# Autodesk Inventor assembly: ModulWalkaNapinajacego
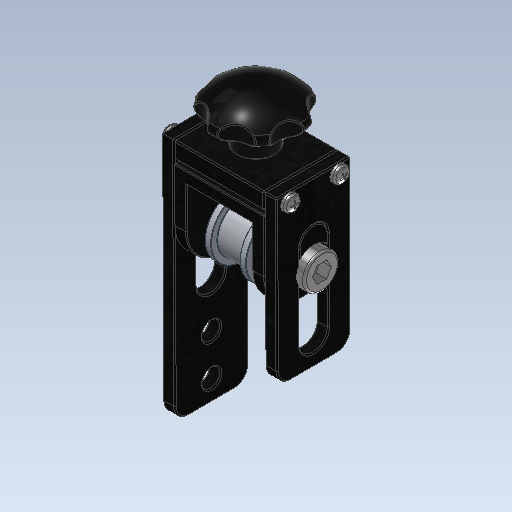
[picture p0: Inventor's stored thumbnail of the model, 512x512]
Saved by Autodesk Inventor 2020 (Build 240168000, 168)
## iProperties
Created: 2020-08-21
Part Number: ModulWalkaNapinajacego
Document SubType Name: Assembly
Designer: estee
Author: estee
## Documents named in this file (9)
- C:\Users\Hesekiel\Desktop\Equatorial-Mount-MUM\Mechanika\Moduł obrotu DEK Bartek\Prawie Gotowe\ModulWalkaNapinajacego.iam
- C:\Users\Hesekiel\Desktop\Equatorial-Mount-MUM\Mechanika\Moduł obrotu DEK Bartek\Prawie Gotowe\Ramka1.ipt
- C:\Users\Hesekiel\Desktop\Equatorial-Mount-MUM\Mechanika\Moduł obrotu DEK Bartek\Prawie Gotowe\Ramka2.ipt
- C:\Users\Hesekiel\Desktop\Equatorial-Mount-MUM\Mechanika\Moduł obrotu DEK Bartek\Prawie Gotowe\Ramka3.ipt
- C:\Users\Hesekiel\Desktop\Equatorial-Mount-MUM\Mechanika\Moduł obrotu DEK Bartek\Prawie Gotowe\Ramka4.ipt
- C:\Users\Hesekiel\Desktop\Equatorial-Mount-MUM\Mechanika\Moduł obrotu DEK Bartek\Prawie Gotowe\EN ISO 7045 - M2 x 6 - 4.8 - H(1).ipt
- C:\Users\Hesekiel\Desktop\Equatorial-Mount-MUM\Mechanika\Moduł obrotu DEK Bartek\Prawie Gotowe\ModulKolaNapinajacego.iam
- C:\Users\Hesekiel\Desktop\Equatorial-Mount-MUM\Mechanika\Moduł obrotu DEK Bartek\Prawie Gotowe\Star Knob M6 Male.ipt
- C:\Users\Hesekiel\Desktop\Equatorial-Mount-MUM\Mechanika\Moduł obrotu DEK Bartek\Prawie Gotowe\ISO 4762 - M5 x 25ISO.ipt
## Components (11 placed, 8 different names)
1. Ramka1:1 — Mate:1, Mate:2, Flush:1, Mate:3, Mate:4, Flush:2, Mate:6, Mate:19, Mate:20, Mate:21, Mate:22
2. Ramka2:1 — Mate:1, Mate:2, Flush:1, Mate:5, Mate:7, Mate:8, Mate:13, Mate:14
3. Ramka3:1 — Mate:3, Mate:4, Flush:2, Mate:9, Mate:10, Mate:11, Mate:12
4. Ramka4:1 — Mate:5, Mate:6, Mate:15, Mate:16
5. BS EN ISO 7045 H - Metric M2 x 6 - 4.8 - H:1 — Mate:7, Mate:13
6. BS EN ISO 7045 H - Metric M2 x 6 - 4.8 - H:2 — Mate:8, Mate:14
7. BS EN ISO 7045 H - Metric M2 x 6 - 4.8 - H:3 — Mate:9, Mate:11
8. BS EN ISO 7045 H - Metric M2 x 6 - 4.8 - H:4 — Mate:10, Mate:12
9. ModulKolaNapinajacego:1 [sub-assembly] — Mate:19, Mate:20
10. Star Knob M6 Male:1 — Mate:15, Mate:16
11. ISO 4762 M5 x 25:1 — Mate:21, Mate:22
## Relationships (22: Mate 20, Flush 2)
- Mate:1: Ramka1:1 ↔ Ramka2:1
- Mate:2: Ramka1:1 ↔ Ramka2:1
- Flush:1: Ramka1:1 ↔ Ramka2:1
- Mate:3: Ramka1:1 ↔ Ramka3:1
- Mate:4: Ramka1:1 ↔ Ramka3:1
- Flush:2: Ramka1:1 ↔ Ramka3:1
- Mate:5: Ramka2:1 ↔ Ramka4:1
- Mate:6: Ramka1:1 ↔ Ramka4:1
- Mate:7: Ramka2:1 ↔ BS EN ISO 7045 H - Metric M2 x 6 - 4.8 - H:1
- Mate:8: Ramka2:1 ↔ BS EN ISO 7045 H - Metric M2 x 6 - 4.8 - H:2
- Mate:9: Ramka3:1 ↔ BS EN ISO 7045 H - Metric M2 x 6 - 4.8 - H:3
- Mate:10: Ramka3:1 ↔ BS EN ISO 7045 H - Metric M2 x 6 - 4.8 - H:4
- Mate:11: Ramka3:1 ↔ BS EN ISO 7045 H - Metric M2 x 6 - 4.8 - H:3
- Mate:12: Ramka3:1 ↔ BS EN ISO 7045 H - Metric M2 x 6 - 4.8 - H:4
- Mate:13: Ramka2:1 ↔ BS EN ISO 7045 H - Metric M2 x 6 - 4.8 - H:1
- Mate:14: Ramka2:1 ↔ BS EN ISO 7045 H - Metric M2 x 6 - 4.8 - H:2
- Mate:15: Ramka4:1 ↔ Star Knob M6 Male:1
- Mate:16: Ramka4:1 ↔ Star Knob M6 Male:1
- Mate:19 (3 mm): Ramka1:1 ↔ ModulKolaNapinajacego:1
- Mate:20: Ramka1:1 ↔ ModulKolaNapinajacego:1
- Mate:21: Ramka1:1 ↔ ISO 4762 M5 x 25:1
- Mate:22: Ramka1:1 ↔ ISO 4762 M5 x 25:1
